# Autodesk Inventor assembly: Передача клиновым ремнем
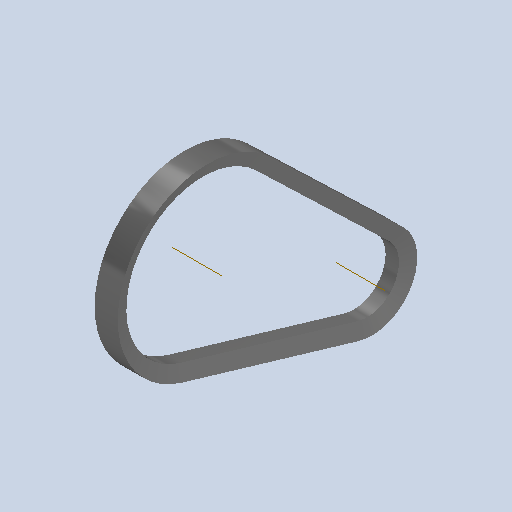
[picture p0: Inventor's stored thumbnail of the model, 512x512]
Saved by Autodesk Inventor 2023 (Build 270158000, 158)
## iProperties
ClientObjectVersion: 1
Created: 2022-05-13
Part Number: Передача клиновым ремнем
Document SubType Name: Assembly
Designer: avkap
Author: avkap
## Documents named in this file (2)
- D:\Стойка\VR-simulator-3D-models\Механизм\Клиновая передача\Мастер проектирования\Передача клиновым ремнем1.iam
- D:\Стойка\VR-simulator-3D-models\Механизм\Клиновая передача\Мастер проектирования\Клиновой ремень1.ipt
## Components (1 placed, 1 different names)
1. Клиновой ремень:1
## Component patterns: (1 elements, first: Клиновой ремень:1)
